# Autodesk Inventor assembly: YAxisIdlerLeft
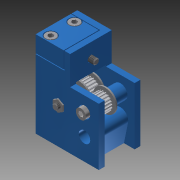
[picture p0: Inventor's stored thumbnail of the model, 180x180]
Saved by Autodesk Inventor 2015 SP1 (Build 190203100, 203)
## iProperties
Created: 2014-08-16
Part Number: YAxisIdlerLeft
Document SubType Name: Assembly
Designer: Jack
Mass: 54.9534 g
Surface Area: 257.859 cm^2
Volume: 35.9784 cm^3
Density: 1.5274 g/cm^3
Author: Jack
Title: Y Idler Left
## Documents named in this file (11)
- C:\Users\Jack\ownCloud\Projects\CrossBot\InventorModel\YAxis\YAxisIdlerLeft.iam
- C:\Users\Jack\ownCloud\Projects\CrossBot\InventorModel\YAxis\YAxisIdler\YIdlerBlockLeft.ipt
- C:\Users\Jack\ownCloud\Projects\CrossBot\InventorModel\YAxis\YAxisIdler\YIdlerCapLeft.ipt
- C:\Users\Jack\ownCloud\Projects\CrossBot\InventorModel\Hardware\Bolts\SHCS\SHCS4\SHCS4x30.ipt
- C:\Users\Jack\ownCloud\Projects\CrossBot\InventorModel\Hardware\Nuts\Nut4.ipt
- C:\Users\Jack\ownCloud\Projects\CrossBot\InventorModel\Hardware\Bolts\SHCS\SHCS4\SHCS4x15.ipt
- C:\Users\Jack\ownCloud\Projects\CrossBot\InventorModel\Hardware\Wahsers\M4Washer.ipt
- C:\Users\Jack\ownCloud\Projects\CrossBot\InventorModel\Hardware\Belt\GT2Idler.iam
- C:\Users\Jack\ownCloud\Projects\CrossBot\InventorModel\YAxis\YAxisBeltIdlerSpacer.ipt
- C:\Users\Jack\ownCloud\Projects\CrossBot\InventorModel\Hardware\Bolts\FHS\FHS4\FHS4x8.ipt
- C:\Users\Jack\ownCloud\Projects\CrossBot\InventorModel\Hardware\Bolts\SHCS\SHCS4\SHCS4x8.ipt
## Components (21 placed, 10 different names)
1. YIdlerBlockLeft:1 — Mate:5, Mate:6, Flush:1, Mate:7, Mate:8, Mate:9, Mate:10, Angle:1, Mate:12, Angle:2, Mate:14, Mate:48, Angle:5, Angle:6, Mate:49, Mate:50, Mate:52, Mate:53, Mate:65, Mate:66, Flush:2, Mate:67, Flush:3, Mate:68, Mate:69, Mate:70, Mate:71
2. YIdlerCapLeft:1 — Mate:15, Mate:16, Mate:17, Mate:18, Mate:71
3. GT2Idler:1 [sub-assembly] — Mate:54, Mate:72, Mate:73
4. GT2Idler:2 [sub-assembly] — Mate:56, Mate:74, Mate:75
5. YAxisBeltIdlerSpacer:1 — Mate:64, Mate:65
6. YAxisBeltIdlerSpacer:2 — Mate:62, Mate:63
7. SHCS4x30:1 — Mate:7, Mate:8, Mate:11, Mate:36, Mate:56, Mate:57, Mate:64
8. SHCS4x30:2 — Mate:9, Mate:10, Mate:13, Mate:35, Mate:54, Mate:60, Mate:62
9. Nut4:2 — Mate:13, Angle:2, Mate:14
10. Nut4:1 — Mate:11, Angle:1, Mate:12
11. M4Washer:4 — Mate:57, Mate:75
12. M4Washer:2 — Mate:35, Mate:52, Mate:73
13. M4Washer:1 — Mate:60, Mate:63, Mate:72
14. M4Washer:3 — Mate:36, Mate:53, Mate:74
15. FHS4x8:1 — Mate:66, Flush:2
16. SHCS4x8:1 — Mate:68, Mate:69
17. FHS4x8:2 — Mate:67, Flush:3
18. SHCS4x15:1 — Mate:15, Mate:18, Mate:19, Mate:70
19. SHCS4x15:2 — Mate:16, Mate:17, Mate:20, Mate:48
20. Nut4:3 — Mate:19, Angle:5, Mate:50
21. Nut4:4 — Mate:20, Angle:6, Mate:49
## Relationships (48: Mate 41, Angle 4, Flush 3)
- Mate:5: YIdlerBlockLeft:1
- Mate:6: YIdlerBlockLeft:1
- Flush:1: YIdlerBlockLeft:1
- Mate:7: YIdlerBlockLeft:1 ↔ SHCS4x30:1
- Mate:8: YIdlerBlockLeft:1 ↔ SHCS4x30:1
- Mate:9: YIdlerBlockLeft:1 ↔ SHCS4x30:2
- Mate:10: YIdlerBlockLeft:1 ↔ SHCS4x30:2
- Mate:11: SHCS4x30:1 ↔ Nut4:1
- Angle:1 (0 deg): YIdlerBlockLeft:1 ↔ Nut4:1
- Mate:12: YIdlerBlockLeft:1 ↔ Nut4:1
- Mate:13: SHCS4x30:2 ↔ Nut4:2
- Angle:2 (0 deg): YIdlerBlockLeft:1 ↔ Nut4:2
- Mate:14: YIdlerBlockLeft:1 ↔ Nut4:2
- Mate:15: YIdlerCapLeft:1 ↔ SHCS4x15:1
- Mate:16: YIdlerCapLeft:1 ↔ SHCS4x15:2
- Mate:17: YIdlerCapLeft:1 ↔ SHCS4x15:2
- Mate:18: YIdlerCapLeft:1 ↔ SHCS4x15:1
- Mate:19: SHCS4x15:1 ↔ Nut4:3
- Mate:20: SHCS4x15:2 ↔ Nut4:4
- Mate:35: SHCS4x30:2 ↔ M4Washer:2
- Mate:36: SHCS4x30:1 ↔ M4Washer:3
- Mate:48: YIdlerBlockLeft:1 ↔ SHCS4x15:2
- Angle:5 (0 deg): YIdlerBlockLeft:1 ↔ Nut4:3
- Angle:6 (0 deg): YIdlerBlockLeft:1 ↔ Nut4:4
- Mate:49: YIdlerBlockLeft:1 ↔ Nut4:4
- Mate:50: YIdlerBlockLeft:1 ↔ Nut4:3
- Mate:52: YIdlerBlockLeft:1 ↔ M4Washer:2
- Mate:53: YIdlerBlockLeft:1 ↔ M4Washer:3
- Mate:54: GT2Idler:1 ↔ SHCS4x30:2
- Mate:56: GT2Idler:2 ↔ SHCS4x30:1
- Mate:57: SHCS4x30:1 ↔ M4Washer:4
- Mate:60: SHCS4x30:2 ↔ M4Washer:1
- Mate:62: YAxisBeltIdlerSpacer:2 ↔ SHCS4x30:2
- Mate:63: YAxisBeltIdlerSpacer:2 ↔ M4Washer:1
- Mate:64: YAxisBeltIdlerSpacer:1 ↔ SHCS4x30:1
- Mate:65: YIdlerBlockLeft:1 ↔ YAxisBeltIdlerSpacer:1
- Mate:66: YIdlerBlockLeft:1 ↔ FHS4x8:1
- Flush:2: YIdlerBlockLeft:1 ↔ FHS4x8:1
- Mate:67: YIdlerBlockLeft:1 ↔ FHS4x8:2
- Flush:3: YIdlerBlockLeft:1 ↔ FHS4x8:2
- Mate:68: YIdlerBlockLeft:1 ↔ SHCS4x8:1
- Mate:69: YIdlerBlockLeft:1 ↔ SHCS4x8:1
- Mate:70: YIdlerBlockLeft:1 ↔ SHCS4x15:1
- Mate:71: YIdlerBlockLeft:1 ↔ YIdlerCapLeft:1
- Mate:72: GT2Idler:1 ↔ M4Washer:1
- Mate:73: GT2Idler:1 ↔ M4Washer:2
- Mate:74: GT2Idler:2 ↔ M4Washer:3
- Mate:75: GT2Idler:2 ↔ M4Washer:4
